# Autodesk Inventor assembly: Assembly2
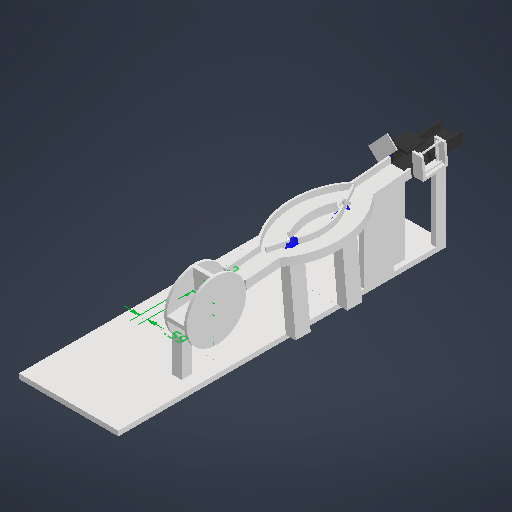
[picture p0: Inventor's stored thumbnail of the model, 512x512]
Saved by Autodesk Inventor 2026.2 (Build 302298000, 298)
## iProperties
Created: 2026-02-23
Part Number: Assembly2
Document SubType Name: Assembly
Designer: danda
Author: danda
## Documents named in this file (14)
- C:\Users\danda\BOM-project\Project\CAD\sorting\Assembly2.iam
- C:\Users\danda\BOM-project\Project\CAD\sorting\stand.ipt
- C:\Users\danda\BOM-project\Project\CAD\sorting\stand2.ipt
- C:\Users\danda\BOM-project\Project\CAD\sorting\inslide.ipt
- C:\Users\danda\BOM-project\Project\CAD\sorting\base.ipt
- C:\Users\danda\BOM-project\Project\CAD\sorting\Towerpro Micro Servo 9g\Towerpro Micro Servo 9g\Towerpro Micro Servo 9g.ipt
- C:\Users\danda\BOM-project\Project\CAD\sorting\motorstand1.ipt
- C:\Users\danda\BOM-project\Project\CAD\sorting\gate.ipt
- C:\Users\danda\BOM-project\Project\CAD\sorting\motorstand2.ipt
- C:\Users\danda\BOM-project\Project\CAD\sorting\gate2.ipt
- C:\Users\danda\BOM-project\Project\CAD\sorting\Sensorroom.ipt
- C:\Users\danda\BOM-project\Project\CAD\sorting\outside3.ipt
- C:\Users\danda\BOM-project\Project\CAD\sorting\wheel.ipt
- C:\Users\danda\BOM-project\Project\CAD\sorting\motorwheelstand.ipt
## Components (20 placed, 13 different names)
1. stand:1 — Mate:5, Flush:8, Mate:30, Mate:51
2. stand2:1 — Mate:4, Flush:1, Flush:7, Mate:17, Mate:18, Mate:30, Mate:31, Mate:32, Flush:13
3. inslide:1 — Flush:8, Mate:17, Mate:18, Mate:31, Mate:32, Flush:13, Flush:18, Mate:42, Flush:20, Flush:21, Mate:52, Flush:28
4. base:1 — Mate:3, Mate:4, Flush:1, Mate:5, Mate:9, Mate:14, Mate:15, Flush:7, Flush:12, Flush:15, Mate:39, Mate:40, Mate:41, Flush:24, Mate:49, Flush:25
5. Towerpro Micro Servo 9g:1 — Mate:11, Mate:12, Mate:13, Insert:1
6. motorstand1:1 — Mate:9, Mate:11, Mate:12, Mate:13, Flush:12, Flush:15
7. gate:1 — Insert:1
8. motorstand2:1 — Mate:21, Mate:22, Mate:23, Mate:39, Mate:40, Mate:41, Flush:31, Mate:56
9. Towerpro Micro Servo 9g:2 — Mate:21, Mate:22, Mate:23, Insert:2, Rotational:1
10. gate2:1 — Insert:2, Rotational:1
11. Sensorroom:1 — Flush:18, Mate:42, Flush:20, Flush:21
12. outside3:1 — Mate:51, Mate:52, Flush:28
13. wheel:1 — Insert:4
14. base:2 — Flush:24, Mate:49, Flush:25, Flush:26, Mate:50, Flush:27, Mate:53
15. base:3 — Flush:26, Mate:50, Flush:27, Mate:60, Flush:32, Flush:33
16. motorstand2:2 — Mate:53, Flush:31, Mate:56, Mate:57, Mate:58, Mate:59
17. Towerpro Micro Servo 9g:3 — Mate:57, Mate:58, Mate:59, Insert:3
18. gate2:3 — Insert:3
19. Towerpro Micro Servo 9g:4 — Mate:61, Mate:62, Mate:63, Insert:4
20. motorwheelstand:1 — Mate:60, Flush:32, Mate:61, Mate:62, Mate:63, Flush:33
## Relationships (56: Mate 34, Flush 17, Insert 4, RevoluteJoint 1)
- Mate:3: base:1
- Mate:4: stand2:1 ↔ base:1
- Flush:1: stand2:1 ↔ base:1
- Mate:5: stand:1 ↔ base:1
- Mate:9: base:1 ↔ motorstand1:1
- Mate:11: Towerpro Micro Servo 9g:1 ↔ motorstand1:1
- Mate:12: Towerpro Micro Servo 9g:1 ↔ motorstand1:1
- Mate:13: Towerpro Micro Servo 9g:1 ↔ motorstand1:1
- Insert:1: Towerpro Micro Servo 9g:1 ↔ gate:1
- Mate:14: base:1
- Mate:15: base:1
- Flush:7: stand2:1 ↔ base:1
- Flush:8: stand:1 ↔ inslide:1
- Mate:17: stand2:1 ↔ inslide:1
- Mate:18: stand2:1 ↔ inslide:1
- Mate:21: motorstand2:1 ↔ Towerpro Micro Servo 9g:2
- Mate:22: motorstand2:1 ↔ Towerpro Micro Servo 9g:2
- Mate:23: motorstand2:1 ↔ Towerpro Micro Servo 9g:2
- Insert:2: Towerpro Micro Servo 9g:2 ↔ gate2:1
- Flush:12 (119.38 mm): base:1 ↔ motorstand1:1
- Mate:30 (85 mm): stand:1 ↔ stand2:1
- Mate:31: stand2:1 ↔ inslide:1
- Mate:32: stand2:1 ↔ inslide:1
- Flush:13: stand2:1 ↔ inslide:1
- Flush:15 (10.16 mm): base:1 ↔ motorstand1:1
- Rotational:1 [RevoluteJoint]: Towerpro Micro Servo 9g:2 ↔ gate2:1
- Mate:39: base:1 ↔ motorstand2:1
- Mate:40: base:1 ↔ motorstand2:1
- Mate:41 (21.336 mm): base:1 ↔ motorstand2:1
- Flush:18: inslide:1 ↔ Sensorroom:1
- Mate:42: inslide:1 ↔ Sensorroom:1
- Flush:20: inslide:1 ↔ Sensorroom:1
- Flush:21: inslide:1 ↔ Sensorroom:1
- Flush:24: base:1 ↔ base:2
- Mate:49: base:1 ↔ base:2
- Flush:25: base:1 ↔ base:2
- Flush:26: base:2 ↔ base:3
- Mate:50: base:2 ↔ base:3
- Flush:27: base:2 ↔ base:3
- Mate:51: stand:1 ↔ outside3:1
- Mate:52: inslide:1 ↔ outside3:1
- Flush:28: inslide:1 ↔ outside3:1
- Mate:53: base:2 ↔ motorstand2:2
- Flush:31: motorstand2:1 ↔ motorstand2:2
- Mate:56 (73.66 mm): motorstand2:1 ↔ motorstand2:2
- Mate:57: motorstand2:2 ↔ Towerpro Micro Servo 9g:3
- Mate:58: motorstand2:2 ↔ Towerpro Micro Servo 9g:3
- Mate:59: motorstand2:2 ↔ Towerpro Micro Servo 9g:3
- Insert:3: Towerpro Micro Servo 9g:3 ↔ gate2:3
- Mate:60: base:3 ↔ motorwheelstand:1
- Flush:32 (24.8666 mm): base:3 ↔ motorwheelstand:1
- Mate:61: Towerpro Micro Servo 9g:4 ↔ motorwheelstand:1
- Mate:62: Towerpro Micro Servo 9g:4 ↔ motorwheelstand:1
- Mate:63: Towerpro Micro Servo 9g:4 ↔ motorwheelstand:1
- Insert:4: wheel:1 ↔ Towerpro Micro Servo 9g:4
- Flush:33 (152.4 mm): base:3 ↔ motorwheelstand:1
## Named parameters: Finish3_Area = 203.593, Finish4_Area = 203.593, Finish5_Area = 203.593
note: some values were not read from the file. Shown as the stored number, unit unknown: "Finish3_Area", "Finish4_Area", "Finish5_Area".
